# Autodesk Inventor assembly: _MK-1_Assembly
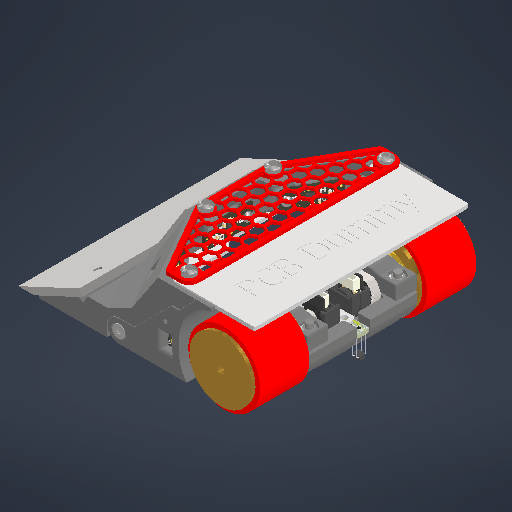
[picture p0: Inventor's stored thumbnail of the model, 512x512]
Saved by Autodesk Inventor 2027 (Build 310192000, 192)
## iProperties
Created: 2026-04-22
Part Number: _MK-1_Assembly
Document SubType Name: Assembly
Designer: Vadim
Author: Vadim
## Documents named in this file (27)
- C:\Users\Vadim\GitHub\NeoSumec\NeoSumec-MiniSumo-MECH\_MK-1_\_MK-1_Assembly.iam
- C:\Users\Vadim\GitHub\NeoSumec\NeoSumec-MiniSumo-MECH\_MK-1_\Models\3D_Print\BodyMotor.ipt
- C:\Users\Vadim\GitHub\NeoSumec\NeoSumec-MiniSumo-MECH\_MK-1_\Models\3D_Print\MotorClamp.ipt
- C:\Users\Vadim\GitHub\NeoSumec\NeoSumec-MiniSumo-MECH\_MK-1_\Models\Metal\pipe.ipt
- C:\Users\Vadim\GitHub\NeoSumec\NeoSumec-MiniSumo-MECH\_MK-1_\Models\Metal\Wheel.ipt
- C:\Users\Vadim\GitHub\NeoSumec\NeoSumec-MiniSumo-MECH\_MK-1_\Models\3rd-party\Pololu Micro Metal Gearmotor 3D (STEP) Models\With Encoder, Side Connector\mmgm-cb-enc-side-con\mmgm-cb-enc-side-con\mmgm-cb-enc-side-con.ipt
- C:\Users\Vadim\GitHub\NeoSumec\NeoSumec-MiniSumo-MECH\_MK-1_\Models\Other technology\silicon bublebum.ipt
- C:\Users\Vadim\GitHub\NeoSumec\NeoSumec-MiniSumo-MECH\_MK-1_\Fasteners\DIN 934 - M3 x 0,5.ipt
- C:\Users\Vadim\GitHub\NeoSumec\NeoSumec-MiniSumo-MECH\_MK-1_\Fasteners\ISO 14580 M3x25-4.8.ipt
- C:\Users\Vadim\GitHub\NeoSumec\NeoSumec-MiniSumo-MECH\_MK-1_\Fasteners\ISO 14581 - M3x16-4.8.ipt
- C:\Users\Vadim\GitHub\NeoSumec\NeoSumec-MiniSumo-MECH\_MK-1_\Fasteners\ISO 14581 - M3x20-4.8.ipt
- C:\Users\Vadim\GitHub\NeoSumec\NeoSumec-MiniSumo-MECH\_MK-1_\Fasteners\DIN 916 - M3  x  6.ipt
- C:\Users\Vadim\GitHub\NeoSumec\NeoSumec-MiniSumo-MECH\_MK-1_\Models\3D_Print\BodyMain.ipt
- C:\Users\Vadim\GitHub\NeoSumec\NeoSumec-MiniSumo-MECH\_MK-1_\Models\3rd-party\pololu-digital-distance-sensor-irs17a\pololu-digital-distance-sensor-irs17a.ipt
- C:\Users\Vadim\GitHub\NeoSumec\NeoSumec-MiniSumo-MECH\_MK-1_\Fasteners\ISO 14583 - M2x5-4.8.ipt
- C:\Users\Vadim\GitHub\NeoSumec\NeoSumec-MiniSumo-MECH\_MK-1_\Fasteners\DIN 562 - M3 x 5,5.ipt
- C:\Users\Vadim\GitHub\NeoSumec\NeoSumec-MiniSumo-MECH\_MK-1_\Fasteners\ISO 14581 - M3x8-4.8.ipt
- C:\Users\Vadim\GitHub\NeoSumec\NeoSumec-MiniSumo-MECH\_MK-1_\Models\PCB\QREBoard_BackSen\QREBoard_BackSen.ipt
- C:\Users\Vadim\GitHub\NeoSumec\NeoSumec-MiniSumo-MECH\_MK-1_\Models\3D_Print\BackSen-TpuPart.ipt
- C:\Users\Vadim\GitHub\NeoSumec\NeoSumec-MiniSumo-MECH\_MK-1_\Models\3D_Print\BodyFront.ipt
- C:\Users\Vadim\GitHub\NeoSumec\NeoSumec-MiniSumo-MECH\_MK-1_\Models\Metal\Knife.ipt
- C:\Users\Vadim\GitHub\NeoSumec\NeoSumec-MiniSumo-MECH\_MK-1_\Fasteners\ISO 14583 - M3x8-4.8.ipt
- C:\Users\Vadim\GitHub\NeoSumec\NeoSumec-MiniSumo-MECH\_MK-1_\Models\PCB\PCBDummy - Main.ipt
- C:\Users\Vadim\GitHub\NeoSumec\NeoSumec-MiniSumo-MECH\_MK-1_\Models\3D_Print\UpperSomething.ipt
- C:\Users\Vadim\GitHub\NeoSumec\NeoSumec-MiniSumo-MECH\_MK-1_\Fasteners\ISO 14583 - M3x4-4.8.ipt
- C:\Users\Vadim\GitHub\NeoSumec\NeoSumec-MiniSumo-MECH\_MK-1_\Models\PCB\PCBDummy - SenRigFront.ipt
- C:\Users\Vadim\GitHub\NeoSumec\NeoSumec-MiniSumo-MECH\_MK-1_\Models\Metal\FrontArmor - Sheet.ipt
## Components (67 placed, 26 different names)
1. Knife:1 — Proti sobě:83, Proti sobě:84, Proti sobě:85
2. BodyFront:1 — Proti sobě:69, Stejný směr:4, Proti sobě:70, Proti sobě:71, Proti sobě:72, Stejný směr:5, Proti sobě:73, Stejný směr:6, Proti sobě:74, Proti sobě:75, Proti sobě:76, Stejný směr:7, Proti sobě:77, Proti sobě:78, Proti sobě:79, Proti sobě:80, Proti sobě:81, Proti sobě:82, Proti sobě:83, Proti sobě:84, Proti sobě:85, Proti sobě:88, Proti sobě:90, Proti sobě:92, Proti sobě:93, Proti sobě:94, Proti sobě:95, Proti sobě:96, Proti sobě:97, Proti sobě:98, Proti sobě:99, Proti sobě:100, Proti sobě:101, Proti sobě:102, Proti sobě:103, Proti sobě:110, Proti sobě:111, Proti sobě:112, Proti sobě:113, Proti sobě:117, Proti sobě:118, Proti sobě:119, Proti sobě:120, Proti sobě:121, Proti sobě:122, Proti sobě:123, Proti sobě:130, Proti sobě:131, Proti sobě:136, Proti sobě:137, Proti sobě:138, Proti sobě:139, Proti sobě:140, Vložit:63, Vložit:64
3. BodyMain:1 — Proti sobě:50, Stejný směr:2, Proti sobě:51, Vložit:53, Proti sobě:52, Vložit:54, Proti sobě:53, Vložit:55, Proti sobě:58, Proti sobě:59, Vložit:56, Proti sobě:60, Vložit:57, Vložit:58, Vložit:59, Vložit:60, Proti sobě:61, Stejný směr:4, Proti sobě:70, Proti sobě:104, Proti sobě:105, Proti sobě:106, Proti sobě:107, Proti sobě:108, Proti sobě:109
4. BodyMotor:1 — Proti sobě:1, Proti sobě:2, Proti sobě:3, Proti sobě:4, Proti sobě:7, Proti sobě:10, Proti sobě:15, Stejný směr:1, Proti sobě:17, Proti sobě:19, Proti sobě:21, Proti sobě:34, Proti sobě:35, Proti sobě:36, Proti sobě:37, Proti sobě:38, Proti sobě:39, Proti sobě:40, Proti sobě:41, Stejný směr:2, Proti sobě:51, Stejný směr:3, Proti sobě:65, Proti sobě:66, Proti sobě:67
5. MotorClamp:1 — Proti sobě:18, Proti sobě:19, Proti sobě:24, Proti sobě:25, Proti sobě:26, Proti sobě:27, Proti sobě:32, Proti sobě:33
6. MotorClamp:2 — Proti sobě:16, Proti sobě:17, Proti sobě:22, Proti sobě:23, Proti sobě:28, Proti sobě:29, Proti sobě:30, Proti sobě:31
7. pipe:1 — Proti sobě:15, Stejný směr:1, Proti sobě:20
8. Wheel:1 — Proti sobě:5, Proti sobě:6, Proti sobě:7, Proti sobě:11, Proti sobě:14, Proti sobě:42, Proti sobě:44
9. Wheel:2 — Proti sobě:8, Proti sobě:9, Proti sobě:10, Proti sobě:12, Proti sobě:13, Proti sobě:45, Proti sobě:46
10. silicon bublebum:1 — Proti sobě:11, Proti sobě:14
11. silicon bublebum:2 — Proti sobě:12, Proti sobě:13
12. UpperSomething:1 — Proti sobě:124, Proti sobě:125, Proti sobě:127, Proti sobě:128, Proti sobě:129, Proti sobě:141
13. mmgm-cb-enc-side-con:1 — Proti sobě:1, Proti sobě:2, Proti sobě:5, Proti sobě:6, Proti sobě:18, Proti sobě:43, Proti sobě:49
14. mmgm-cb-enc-side-con:2 — Proti sobě:3, Proti sobě:4, Proti sobě:8, Proti sobě:9, Proti sobě:16, Proti sobě:47, Proti sobě:48
15. pololu-digital-distance-sensor-irs17a:1 — Vložit:53, Proti sobě:52, Proti sobě:54, Proti sobě:55
16. pololu-digital-distance-sensor-irs17a:2 — Vložit:54, Proti sobě:53, Proti sobě:56, Proti sobě:57
17. pololu-digital-distance-sensor-irs17a:3 — Proti sobě:71, Proti sobě:72, Stejný směr:5, Proti sobě:86, Proti sobě:87
18. pololu-digital-distance-sensor-irs17a:4 — Proti sobě:73, Stejný směr:6, Proti sobě:74, Proti sobě:89
19. pololu-digital-distance-sensor-irs17a:5 — Proti sobě:75, Proti sobě:76, Stejný směr:7, Proti sobě:91
20. QREBoard_BackSen:1 — Stejný směr:3, Vložit:61
21. PCBDummy - Main:1 — Proti sobě:121, Proti sobě:122, Proti sobě:123
22. PCBDummy - SenRigFront:1 — Proti sobě:132, Proti sobě:133, Proti sobě:134, Proti sobě:135, Proti sobě:136
23. BackSen-TpuPart:1 — Proti sobě:66, Proti sobě:67, Vložit:61, Proti sobě:68
24. FrontArmor - Sheet:1 — Vložit:63, Vložit:64, Proti sobě:141
25. DIN 916 - M3  x  6:1 — Proti sobě:42, Proti sobě:43
26. DIN 916 - M3  x  6:2 — Proti sobě:44, Proti sobě:49
27. DIN 916 - M3  x  6:3 — Proti sobě:45, Proti sobě:47
28. DIN 916 - M3  x  6:4 — Proti sobě:46, Proti sobě:48
29. ISO 14581 - M3x16-4.8:1 — Proti sobě:36, Proti sobě:37
30. ISO 14581 - M3x16-4.8:2 — Proti sobě:38, Proti sobě:39
31. ISO 14581 - M3x20-4.8:1 — Proti sobě:34, Proti sobě:35
32. ISO 14581 - M3x20-4.8:2 — Proti sobě:40, Proti sobě:41
33. DIN 934 - M3 x 0,5:1 — Proti sobě:25, Proti sobě:26, Proti sobě:33
34. DIN 934 - M3 x 0,5:2 — Proti sobě:24, Proti sobě:27, Proti sobě:32
35. DIN 934 - M3 x 0,5:3 — Proti sobě:22, Proti sobě:29, Proti sobě:30
36. DIN 934 - M3 x 0,5:4 — Proti sobě:23, Proti sobě:28, Proti sobě:31
37. DIN 934 - M3 x 0,5:5 — Vložit:60, Proti sobě:61
38. DIN 562 - M3 x 5,5:1 — Vložit:55, Proti sobě:58
39. ISO 14580 M3x25-4.8:1 — Proti sobě:20, Proti sobě:21, Proti sobě:50
40. DIN 934 - M3 x 0,5:9 — Proti sobě:104, Proti sobě:105, Proti sobě:106
41. DIN 934 - M3 x 0,5:10 — Proti sobě:107, Proti sobě:108, Proti sobě:109
42. ISO 14583 - M3x8-4.8:1 — Proti sobě:110, Proti sobě:111
43. ISO 14583 - M3x8-4.8:2 — Proti sobě:112, Proti sobě:113
44. ISO 14581 - M3x8-4.8:1 — Vložit:58, Proti sobě:69
45. ISO 14581 - M3x8-4.8:2 — Vložit:59
46. DIN 562 - M3 x 5,5:2 — Proti sobě:59, Vložit:56
47. DIN 562 - M3 x 5,5:3 — Proti sobě:60, Vložit:57
48. ISO 14581 - M3x8-4.8:4 — Proti sobě:102, Proti sobě:103
49. ISO 14581 - M3x8-4.8:5 — Proti sobě:100, Proti sobě:101
50. ISO 14581 - M3x8-4.8:6 — Proti sobě:98, Proti sobě:99
51. DIN 562 - M3 x 5,5:4 — Proti sobě:95, Proti sobě:96, Proti sobě:97, Proti sobě:137, Proti sobě:138
52. DIN 562 - M3 x 5,5:5 — Proti sobě:92, Proti sobě:93, Proti sobě:94, Proti sobě:139, Proti sobě:140
53. ISO 14583 - M3x8-4.8:3 — Proti sobě:117, Proti sobě:128
54. ISO 14583 - M3x8-4.8:4 — Proti sobě:118, Proti sobě:124, Proti sobě:127
55. DIN 934 - M3 x 0,5:6 — Vložit:62, Proti sobě:68
56. ISO 14581 - M3x8-4.8:3 — Proti sobě:65, Vložit:62
57. ISO 14583 - M2x5-4.8:1 — Proti sobě:54, Proti sobě:55
58. ISO 14583 - M2x5-4.8:2 — Proti sobě:56, Proti sobě:57
59. ISO 14583 - M2x5-4.8:3 — Proti sobě:86, Proti sobě:87
60. ISO 14583 - M2x5-4.8:4 — Proti sobě:88, Proti sobě:89
61. ISO 14583 - M2x5-4.8:5 — Proti sobě:90, Proti sobě:91
62. ISO 14583 - M3x4-4.8:1 — Proti sobě:130, Proti sobě:133, Proti sobě:135
63. ISO 14583 - M3x4-4.8:2 — Proti sobě:131, Proti sobě:132, Proti sobě:134
64. ISO 14583 - M3x8-4.8:5 — Proti sobě:119
65. ISO 14583 - M3x8-4.8:6 — Proti sobě:120, Proti sobě:125, Proti sobě:129
66. DIN 934 - M3 x 0,5:7 — Proti sobě:77, Proti sobě:78, Proti sobě:79
67. DIN 934 - M3 x 0,5:8 — Proti sobě:80, Proti sobě:81, Proti sobě:82
## Relationships (153: Mate 134, Insert 12, Flush 7)
- Proti sobě:1 [Mate]: BodyMotor:1 ↔ mmgm-cb-enc-side-con:1
- Proti sobě:2 [Mate] (0.125 mm): BodyMotor:1 ↔ mmgm-cb-enc-side-con:1
- Proti sobě:3 [Mate]: BodyMotor:1 ↔ mmgm-cb-enc-side-con:2
- Proti sobě:4 [Mate] (0.125 mm): BodyMotor:1 ↔ mmgm-cb-enc-side-con:2
- Proti sobě:5 [Mate]: Wheel:1 ↔ mmgm-cb-enc-side-con:1
- Proti sobě:6 [Mate] (0.1 mm): Wheel:1 ↔ mmgm-cb-enc-side-con:1
- Proti sobě:7 [Mate] (0.25 mm): BodyMotor:1 ↔ Wheel:1
- Proti sobě:8 [Mate]: Wheel:2 ↔ mmgm-cb-enc-side-con:2
- Proti sobě:9 [Mate] (0.15 mm): Wheel:2 ↔ mmgm-cb-enc-side-con:2
- Proti sobě:10 [Mate] (0.25 mm): BodyMotor:1 ↔ Wheel:2
- Proti sobě:11 [Mate]: Wheel:1 ↔ silicon bublebum:1
- Proti sobě:12 [Mate]: Wheel:2 ↔ silicon bublebum:2
- Proti sobě:13 [Mate]: Wheel:2 ↔ silicon bublebum:2
- Proti sobě:14 [Mate]: Wheel:1 ↔ silicon bublebum:1
- Proti sobě:15 [Mate]: BodyMotor:1 ↔ pipe:1
- Stejný směr:1 [Flush]: BodyMotor:1 ↔ pipe:1
- Proti sobě:16 [Mate]: MotorClamp:2 ↔ mmgm-cb-enc-side-con:2
- Proti sobě:17 [Mate]: BodyMotor:1 ↔ MotorClamp:2
- Proti sobě:18 [Mate]: MotorClamp:1 ↔ mmgm-cb-enc-side-con:1
- Proti sobě:19 [Mate]: BodyMotor:1 ↔ MotorClamp:1
- Proti sobě:20 [Mate]: pipe:1 ↔ ISO 14580 M3x25-4.8:1
- Proti sobě:21 [Mate]: BodyMotor:1 ↔ ISO 14580 M3x25-4.8:1
- Proti sobě:22 [Mate]: MotorClamp:2 ↔ DIN 934 - M3 x 0,5:3
- Proti sobě:23 [Mate]: MotorClamp:2 ↔ DIN 934 - M3 x 0,5:4
- Proti sobě:24 [Mate]: MotorClamp:1 ↔ DIN 934 - M3 x 0,5:2
- Proti sobě:25 [Mate]: MotorClamp:1 ↔ DIN 934 - M3 x 0,5:1
- Proti sobě:26 [Mate] (0.1 mm): MotorClamp:1 ↔ DIN 934 - M3 x 0,5:1
- Proti sobě:27 [Mate] (0.1 mm): MotorClamp:1 ↔ DIN 934 - M3 x 0,5:2
- Proti sobě:28 [Mate] (0.1 mm): MotorClamp:2 ↔ DIN 934 - M3 x 0,5:4
- Proti sobě:29 [Mate] (0.1 mm): MotorClamp:2 ↔ DIN 934 - M3 x 0,5:3
- Proti sobě:30 [Mate]: MotorClamp:2 ↔ DIN 934 - M3 x 0,5:3
- Proti sobě:31 [Mate]: MotorClamp:2 ↔ DIN 934 - M3 x 0,5:4
- Proti sobě:32 [Mate]: MotorClamp:1 ↔ DIN 934 - M3 x 0,5:2
- Proti sobě:33 [Mate]: MotorClamp:1 ↔ DIN 934 - M3 x 0,5:1
- Proti sobě:34 [Mate]: BodyMotor:1 ↔ ISO 14581 - M3x20-4.8:1
- Proti sobě:35 [Mate]: BodyMotor:1 ↔ ISO 14581 - M3x20-4.8:1
- Proti sobě:36 [Mate]: BodyMotor:1 ↔ ISO 14581 - M3x16-4.8:1
- Proti sobě:37 [Mate]: BodyMotor:1 ↔ ISO 14581 - M3x16-4.8:1
- Proti sobě:38 [Mate]: BodyMotor:1 ↔ ISO 14581 - M3x16-4.8:2
- Proti sobě:39 [Mate]: BodyMotor:1 ↔ ISO 14581 - M3x16-4.8:2
- Proti sobě:40 [Mate]: BodyMotor:1 ↔ ISO 14581 - M3x20-4.8:2
- Proti sobě:41 [Mate]: BodyMotor:1 ↔ ISO 14581 - M3x20-4.8:2
- Proti sobě:42 [Mate]: Wheel:1 ↔ DIN 916 - M3  x  6:1
- Proti sobě:43 [Mate]: mmgm-cb-enc-side-con:1 ↔ DIN 916 - M3  x  6:1
- Proti sobě:44 [Mate]: Wheel:1 ↔ DIN 916 - M3  x  6:2
- Proti sobě:45 [Mate]: Wheel:2 ↔ DIN 916 - M3  x  6:3
- Proti sobě:46 [Mate]: Wheel:2 ↔ DIN 916 - M3  x  6:4
- Proti sobě:47 [Mate]: mmgm-cb-enc-side-con:2 ↔ DIN 916 - M3  x  6:3
- Proti sobě:48 [Mate]: mmgm-cb-enc-side-con:2 ↔ DIN 916 - M3  x  6:4
- Proti sobě:49 [Mate]: mmgm-cb-enc-side-con:1 ↔ DIN 916 - M3  x  6:2
- Proti sobě:50 [Mate]: BodyMain:1 ↔ ISO 14580 M3x25-4.8:1
- Stejný směr:2 [Flush]: BodyMain:1 ↔ BodyMotor:1
- Proti sobě:51 [Mate] (0.5 mm): BodyMain:1 ↔ BodyMotor:1
- Vložit:53 [Insert]: BodyMain:1 ↔ pololu-digital-distance-sensor-irs17a:1
- Proti sobě:52 [Mate]: BodyMain:1 ↔ pololu-digital-distance-sensor-irs17a:1
- Vložit:54 [Insert]: BodyMain:1 ↔ pololu-digital-distance-sensor-irs17a:2
- Proti sobě:53 [Mate]: BodyMain:1 ↔ pololu-digital-distance-sensor-irs17a:2
- Proti sobě:54 [Mate]: pololu-digital-distance-sensor-irs17a:1 ↔ ISO 14583 - M2x5-4.8:1
- Proti sobě:55 [Mate]: pololu-digital-distance-sensor-irs17a:1 ↔ ISO 14583 - M2x5-4.8:1
- Proti sobě:56 [Mate]: pololu-digital-distance-sensor-irs17a:2 ↔ ISO 14583 - M2x5-4.8:2
- Proti sobě:57 [Mate]: pololu-digital-distance-sensor-irs17a:2 ↔ ISO 14583 - M2x5-4.8:2
- Vložit:55 [Insert]: BodyMain:1 ↔ DIN 562 - M3 x 5,5:1
- Proti sobě:58 [Mate]: BodyMain:1 ↔ DIN 562 - M3 x 5,5:1
- Proti sobě:59 [Mate] (0.075 mm): BodyMain:1 ↔ DIN 562 - M3 x 5,5:2
- Vložit:56 [Insert]: BodyMain:1 ↔ DIN 562 - M3 x 5,5:2
- Proti sobě:60 [Mate] (0.075 mm): BodyMain:1 ↔ DIN 562 - M3 x 5,5:3
- Vložit:57 [Insert]: BodyMain:1 ↔ DIN 562 - M3 x 5,5:3
- Vložit:58 [Insert]: BodyMain:1 ↔ ISO 14581 - M3x8-4.8:1
- Vložit:59 [Insert]: BodyMain:1 ↔ ISO 14581 - M3x8-4.8:2
- Vložit:60 [Insert]: BodyMain:1 ↔ DIN 934 - M3 x 0,5:5
- Proti sobě:61 [Mate]: BodyMain:1 ↔ DIN 934 - M3 x 0,5:5
- Stejný směr:3 [Flush]: BodyMotor:1 ↔ QREBoard_BackSen:1
- Proti sobě:65 [Mate]: BodyMotor:1 ↔ ISO 14581 - M3x8-4.8:3
- Proti sobě:66 [Mate]: BodyMotor:1 ↔ BackSen-TpuPart:1
- Proti sobě:67 [Mate]: BodyMotor:1 ↔ BackSen-TpuPart:1
- Vložit:61 [Insert]: QREBoard_BackSen:1 ↔ BackSen-TpuPart:1
- Vložit:62 [Insert]: DIN 934 - M3 x 0,5:6 ↔ ISO 14581 - M3x8-4.8:3
- Proti sobě:68 [Mate]: BackSen-TpuPart:1 ↔ DIN 934 - M3 x 0,5:6
- Proti sobě:69 [Mate]: BodyFront:1 ↔ ISO 14581 - M3x8-4.8:1
- Stejný směr:4 [Flush]: BodyFront:1 ↔ BodyMain:1
- Proti sobě:70 [Mate]: BodyFront:1 ↔ BodyMain:1
- Proti sobě:71 [Mate]: BodyFront:1 ↔ pololu-digital-distance-sensor-irs17a:3
- Proti sobě:72 [Mate]: BodyFront:1 ↔ pololu-digital-distance-sensor-irs17a:3
- Stejný směr:5 [Flush]: BodyFront:1 ↔ pololu-digital-distance-sensor-irs17a:3
- Proti sobě:73 [Mate]: BodyFront:1 ↔ pololu-digital-distance-sensor-irs17a:4
- Stejný směr:6 [Flush]: BodyFront:1 ↔ pololu-digital-distance-sensor-irs17a:4
- Proti sobě:74 [Mate]: BodyFront:1 ↔ pololu-digital-distance-sensor-irs17a:4
- Proti sobě:75 [Mate]: BodyFront:1 ↔ pololu-digital-distance-sensor-irs17a:5
- Proti sobě:76 [Mate]: BodyFront:1 ↔ pololu-digital-distance-sensor-irs17a:5
- Stejný směr:7 [Flush]: BodyFront:1 ↔ pololu-digital-distance-sensor-irs17a:5
- Proti sobě:77 [Mate]: BodyFront:1 ↔ DIN 934 - M3 x 0,5:7
- Proti sobě:78 [Mate]: BodyFront:1 ↔ DIN 934 - M3 x 0,5:7
- Proti sobě:79 [Mate]: BodyFront:1 ↔ DIN 934 - M3 x 0,5:7
- Proti sobě:80 [Mate]: BodyFront:1 ↔ DIN 934 - M3 x 0,5:8
- Proti sobě:81 [Mate]: BodyFront:1 ↔ DIN 934 - M3 x 0,5:8
- Proti sobě:82 [Mate]: BodyFront:1 ↔ DIN 934 - M3 x 0,5:8
- Proti sobě:83 [Mate]: Knife:1 ↔ BodyFront:1
- Proti sobě:84 [Mate]: Knife:1 ↔ BodyFront:1
- Proti sobě:85 [Mate]: Knife:1 ↔ BodyFront:1
- Proti sobě:86 [Mate]: pololu-digital-distance-sensor-irs17a:3 ↔ ISO 14583 - M2x5-4.8:3
- Proti sobě:87 [Mate]: pololu-digital-distance-sensor-irs17a:3 ↔ ISO 14583 - M2x5-4.8:3
- Proti sobě:88 [Mate]: BodyFront:1 ↔ ISO 14583 - M2x5-4.8:4
- Proti sobě:89 [Mate]: pololu-digital-distance-sensor-irs17a:4 ↔ ISO 14583 - M2x5-4.8:4
- Proti sobě:90 [Mate]: BodyFront:1 ↔ ISO 14583 - M2x5-4.8:5
- Proti sobě:91 [Mate]: pololu-digital-distance-sensor-irs17a:5 ↔ ISO 14583 - M2x5-4.8:5
- Proti sobě:92 [Mate]: BodyFront:1 ↔ DIN 562 - M3 x 5,5:5
- Proti sobě:93 [Mate]: BodyFront:1 ↔ DIN 562 - M3 x 5,5:5
- Proti sobě:94 [Mate]: BodyFront:1 ↔ DIN 562 - M3 x 5,5:5
- Proti sobě:95 [Mate]: BodyFront:1 ↔ DIN 562 - M3 x 5,5:4
- Proti sobě:96 [Mate]: BodyFront:1 ↔ DIN 562 - M3 x 5,5:4
- Proti sobě:97 [Mate]: BodyFront:1 ↔ DIN 562 - M3 x 5,5:4
- Proti sobě:98 [Mate]: BodyFront:1 ↔ ISO 14581 - M3x8-4.8:6
- Proti sobě:99 [Mate]: BodyFront:1 ↔ ISO 14581 - M3x8-4.8:6
- Proti sobě:100 [Mate]: BodyFront:1 ↔ ISO 14581 - M3x8-4.8:5
- Proti sobě:101 [Mate]: BodyFront:1 ↔ ISO 14581 - M3x8-4.8:5
- Proti sobě:102 [Mate]: BodyFront:1 ↔ ISO 14581 - M3x8-4.8:4
- Proti sobě:103 [Mate]: BodyFront:1 ↔ ISO 14581 - M3x8-4.8:4
- Proti sobě:104 [Mate]: BodyMain:1 ↔ DIN 934 - M3 x 0,5:9
- Proti sobě:105 [Mate]: BodyMain:1 ↔ DIN 934 - M3 x 0,5:9
- Proti sobě:106 [Mate]: BodyMain:1 ↔ DIN 934 - M3 x 0,5:9
- Proti sobě:107 [Mate]: BodyMain:1 ↔ DIN 934 - M3 x 0,5:10
- Proti sobě:108 [Mate]: BodyMain:1 ↔ DIN 934 - M3 x 0,5:10
- Proti sobě:109 [Mate]: BodyMain:1 ↔ DIN 934 - M3 x 0,5:10
- Proti sobě:110 [Mate]: BodyFront:1 ↔ ISO 14583 - M3x8-4.8:1
- Proti sobě:111 [Mate]: BodyFront:1 ↔ ISO 14583 - M3x8-4.8:1
- Proti sobě:112 [Mate]: BodyFront:1 ↔ ISO 14583 - M3x8-4.8:2
- Proti sobě:113 [Mate]: BodyFront:1 ↔ ISO 14583 - M3x8-4.8:2
- Proti sobě:117 [Mate]: BodyFront:1 ↔ ISO 14583 - M3x8-4.8:3
- Proti sobě:118 [Mate]: BodyFront:1 ↔ ISO 14583 - M3x8-4.8:4
- Proti sobě:119 [Mate]: BodyFront:1 ↔ ISO 14583 - M3x8-4.8:5
- Proti sobě:120 [Mate]: BodyFront:1 ↔ ISO 14583 - M3x8-4.8:6
- Proti sobě:121 [Mate]: BodyFront:1 ↔ PCBDummy - Main:1
- Proti sobě:122 [Mate]: BodyFront:1 ↔ PCBDummy - Main:1
- Proti sobě:123 [Mate]: BodyFront:1 ↔ PCBDummy - Main:1
- Proti sobě:124 [Mate]: UpperSomething:1 ↔ ISO 14583 - M3x8-4.8:4
- Proti sobě:125 [Mate]: UpperSomething:1 ↔ ISO 14583 - M3x8-4.8:6
- Proti sobě:127 [Mate]: UpperSomething:1 ↔ ISO 14583 - M3x8-4.8:4
- Proti sobě:128 [Mate]: UpperSomething:1 ↔ ISO 14583 - M3x8-4.8:3
- Proti sobě:129 [Mate]: UpperSomething:1 ↔ ISO 14583 - M3x8-4.8:6
- Proti sobě:130 [Mate]: BodyFront:1 ↔ ISO 14583 - M3x4-4.8:1
- Proti sobě:131 [Mate]: BodyFront:1 ↔ ISO 14583 - M3x4-4.8:2
- Proti sobě:132 [Mate]: PCBDummy - SenRigFront:1 ↔ ISO 14583 - M3x4-4.8:2
- Proti sobě:133 [Mate]: PCBDummy - SenRigFront:1 ↔ ISO 14583 - M3x4-4.8:1
- Proti sobě:134 [Mate]: PCBDummy - SenRigFront:1 ↔ ISO 14583 - M3x4-4.8:2
- Proti sobě:135 [Mate]: PCBDummy - SenRigFront:1 ↔ ISO 14583 - M3x4-4.8:1
- Proti sobě:136 [Mate]: BodyFront:1 ↔ PCBDummy - SenRigFront:1
- Proti sobě:137 [Mate]: BodyFront:1 ↔ DIN 562 - M3 x 5,5:4
- Proti sobě:138 [Mate]: BodyFront:1 ↔ DIN 562 - M3 x 5,5:4
- Proti sobě:139 [Mate]: BodyFront:1 ↔ DIN 562 - M3 x 5,5:5
- Proti sobě:140 [Mate]: BodyFront:1 ↔ DIN 562 - M3 x 5,5:5
- Vložit:63 [Insert]: BodyFront:1 ↔ FrontArmor - Sheet:1
- Vložit:64 [Insert]: BodyFront:1 ↔ FrontArmor - Sheet:1
- Proti sobě:141 [Mate]: UpperSomething:1 ↔ FrontArmor - Sheet:1
